# Autodesk Inventor assembly: Assemblyzomman
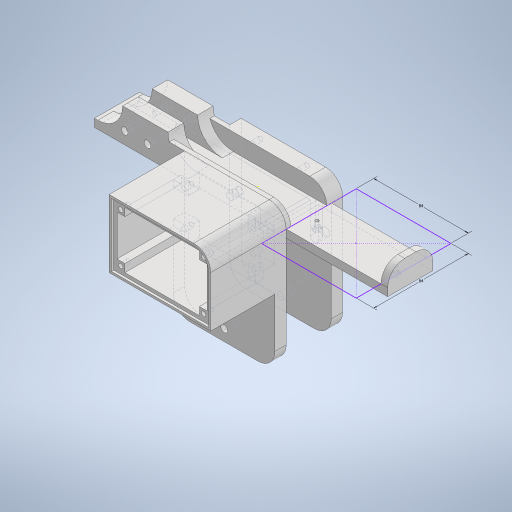
[picture p0: Inventor's stored thumbnail of the model, 512x512]
Saved by Autodesk Inventor 2024.2 (Build 282272000, 272)
## iProperties
Created: 2023-11-10
Part Number: Assemblyzomman
Document SubType Name: Assembly
Designer: Rene
Author: Rene
## Documents named in this file (3)
- C:\Users\Pieber\OneDrive - HTL Weiz\2023.24\Labor\Bergler\Zeitmessung\Halterung_Lichtschranke\Zeitmessung_Lichtschranke_Halterung.iam
- C:\Users\Pieber\OneDrive - HTL Weiz\2023.24\Labor\Bergler\Zeitmessung\Halterung_Lichtschranke\Zeitmessung_Halterung.ipt
- C:\Users\Pieber\OneDrive - HTL Weiz\2023.24\Labor\Bergler\Zeitmessung\Halterung_Lichtschranke\Gehäuse.ipt
## Components (2 placed, 2 different names)
1. Zeitmessung_Halterung:1 — Starr:1
2. Gehäuse:1 — Starr:1
## Relationships (1: WeldJoint 1)
- Starr:1 [WeldJoint]: Zeitmessung_Halterung:1 ↔ Gehäuse:1
